# Autodesk Inventor assembly: Electromanetic brake
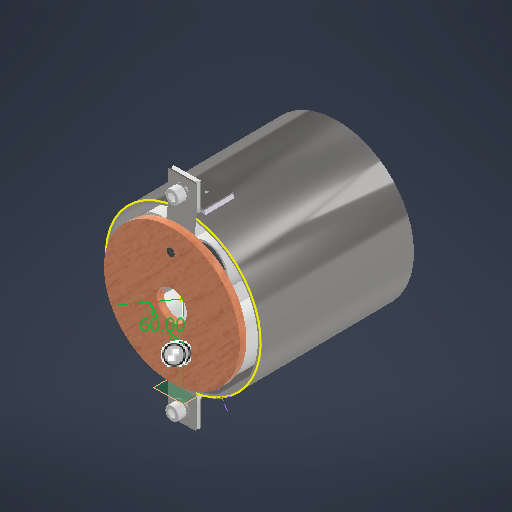
[picture p0: Inventor's stored thumbnail of the model, 512x512]
Saved by Autodesk Inventor 2026.3 (Build 303398000, 398)
## iProperties
Created: 2026-08-09
Part Number: Electromanetic brake
Document SubType Name: Assembly
Designer: matot
Author: matot
## Documents named in this file (8)
- C:\Users\matot\OneDrive - Stellenbosch University\2026\MechatronicsProject478\Building the joint\Joint Assembly\Drawings\Electromanetic brake.iam
- C:\Users\matot\OneDrive - Stellenbosch University\2026\MechatronicsProject478\Building the joint\Joint Assembly\Electromagnet final_key.iam
- C:\Users\matot\OneDrive - Stellenbosch University\2026\MechatronicsProject478\Building the joint\Joint Assembly\Pressure platform.ipt
- C:\Users\matot\OneDrive - Stellenbosch University\2026\MechatronicsProject478\Building the joint\Joint Assembly\din_912-m6x1-10-10_9.ipt
- C:\Users\matot\OneDrive - Stellenbosch University\Documents\Inventor\Content Center Files\R2026\en-US\ISO 7089\ISO 7089 - 6 - 140 HV(1).ipt
- C:\Users\matot\OneDrive - Stellenbosch University\2026\MechatronicsProject478\Building the joint\Joint Assembly\Friction Plate.ipt
- C:\Users\matot\OneDrive - Stellenbosch University\Documents\Inventor\Content Center Files\R2026\en-US\ISO 4035(2)\ISO 4035 - M4 - ISO.ipt
- C:\Users\matot\OneDrive - Stellenbosch University\Documents\Inventor\Content Center Files\R2026\en-US\ISO 7046-1 H(1)\ISO 7046-1 - M3 x 4_ - 4.8 - H - ISO.ipt
## Components (12 placed, 7 different names)
1. Electromagnet final_key:1 [sub-assembly] — Mate:1, Insert:1, Flush:1, Flush:2, Mate:2, Insert:2, Flush:3, Flush:4, Insert:7
2. Pressure platform:1 — Mate:1, Insert:1, Flush:1, Flush:2, Insert:4, Mate:6, Mate:7
3. Pressure platform:2 — Mate:2, Insert:2, Flush:3, Flush:4, Insert:3, Insert:8
4. din_912-m6x1-10-10_9:1 — Insert:5
5. din_912-m6x1-10-10_9:2 — Insert:6
6. ISO 7089 6:1 — Insert:3, Insert:6
7. ISO 7089 6:2 — Insert:4, Insert:5
8. Friction Plate:1 — Insert:7, Insert:9, Mate:3, Mate:4
9. ISO 4035 M4:1 — Insert:8
10. ISO 4035 M4:2 — Insert:9, Mate:5, Mate:6, Mate:7
11. ISO 7046-1 H M3 x 4 - 4.8 - H:1 — Mate:3
12. ISO 7046-1 H M3 x 4 - 4.8 - H:2 — Mate:4, Mate:5
## Relationships (20: Insert 9, Mate 7, Flush 4)
- Mate:1: Electromagnet final_key:1 ↔ Pressure platform:1
- Insert:1: Electromagnet final_key:1 ↔ Pressure platform:1
- Flush:1: Electromagnet final_key:1 ↔ Pressure platform:1
- Flush:2: Electromagnet final_key:1 ↔ Pressure platform:1
- Mate:2: Electromagnet final_key:1 ↔ Pressure platform:2
- Insert:2: Electromagnet final_key:1 ↔ Pressure platform:2
- Flush:3: Electromagnet final_key:1 ↔ Pressure platform:2
- Flush:4: Electromagnet final_key:1 ↔ Pressure platform:2
- Insert:3: Pressure platform:2 ↔ ISO 7089 6:1
- Insert:4: Pressure platform:1 ↔ ISO 7089 6:2
- Insert:5: din_912-m6x1-10-10_9:1 ↔ ISO 7089 6:2
- Insert:6: din_912-m6x1-10-10_9:2 ↔ ISO 7089 6:1
- Insert:7 (103.5 mm): Electromagnet final_key:1 ↔ Friction Plate:1
- Insert:8: Pressure platform:2 ↔ ISO 4035 M4:1
- Insert:9: Friction Plate:1 ↔ ISO 4035 M4:2
- Mate:3: Friction Plate:1 ↔ ISO 7046-1 H M3 x 4 - 4.8 - H:1
- Mate:4: Friction Plate:1 ↔ ISO 7046-1 H M3 x 4 - 4.8 - H:2
- Mate:5: ISO 4035 M4:2 ↔ ISO 7046-1 H M3 x 4 - 4.8 - H:2
- Mate:6: Pressure platform:1 ↔ ISO 4035 M4:2
- Mate:7: Pressure platform:1 ↔ ISO 4035 M4:2
